# Autodesk Inventor assembly: Assembly-PCB alone
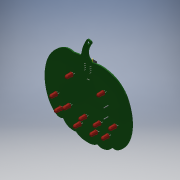
[picture p0: Inventor's stored thumbnail of the model, 180x180]
Saved by Autodesk Inventor 2018 (Build 220112000, 112)
## iProperties
Created: 2019-08-14
Part Number: Assembly-PCB alone
Document SubType Name: Assembly
Designer: Jamal Bouajjaj
Author: Jamal Bouajjaj
## iProperties of the stored document C_1206_3216Metric.iam
Created: 2019-10-04
Part Number: C_1206_3216Metric
Document SubType Name: Assembly
Designer: Electro707
Author: Electro707
## iProperties of the stored document SOLID.ipt
Created: 2019-10-04
Part Number: SOLID
Material: Generic
Document SubType Name: Modeling
Designer: Electro707
Density: 1 g/cm^3
Appearance: Default
Mass: 0.155302 g
Surface Area: 1.85065 cm^2
Volume: 0.155302 cm^3
Author: Electro707
## iProperties of the stored document BC2AAPC.iam
Created: 2019-10-04
Part Number: BC2AAPC
Document SubType Name: Assembly
Designer: Electro707
Author: Electro707
## iProperties of the stored document SOLID_2.ipt
Created: 2019-08-14
Part Number: SOLID_2
Material: Generic
Document SubType Name: Modeling
Designer: Jamal Bouajjaj
Density: 1 g/cm^3
Appearance: Default
Author: Jamal Bouajjaj
## iProperties of the stored document COMPOUND.ipt
Created: 2019-08-14
Part Number: COMPOUND
Material: Generic
Document SubType Name: Modeling
Designer: Jamal Bouajjaj
Density: 1 g/cm^3
Appearance: Default
Mass: 6.62606 g
Surface Area: 82.2116 cm^2
Volume: 6.62606 cm^3
Author: Jamal Bouajjaj
## iProperties of the stored document DIP-8_W7.62mm_Socket.iam
Created: 2019-08-14
Part Number: DIP-8_W7.62mm_Socket
Document SubType Name: Assembly
Designer: Jamal Bouajjaj
Author: Jamal Bouajjaj
## iProperties of the stored document SOLID_4.ipt
Created: 2019-08-14
Part Number: SOLID_4
Material: Generic
Document SubType Name: Modeling
Designer: Jamal Bouajjaj
Density: 1 g/cm^3
Appearance: Default
Mass: 0.075906 g
Surface Area: 1.25578 cm^2
Volume: 0.075906 cm^3
Author: Jamal Bouajjaj
## iProperties of the stored document SOLID_1.ipt
Created: 2019-08-14
Part Number: SOLID_1
Material: Generic
Document SubType Name: Modeling
Designer: Jamal Bouajjaj
Density: 1 g/cm^3
Appearance: Default
Author: Jamal Bouajjaj
## iProperties of the stored document DIP-8_W7.62mm.ipt
Company: FreeCAD
Created: 2017-03-07
Part Number: DIP-8_W7.62mm
Material: Generic
Description: model of DIP-8_W7.62mm
Document SubType Name: Modeling
Designer: Jamal Bouajjaj
Density: 1 g/cm^3
Appearance: Default
Mass: 0.184953 g
Surface Area: 2.97438 cm^2
Volume: 0.184953 cm^3
Sending System: kicad StepUp
Preprocessor: OCC
Title: DIP-8_W7.62mm.step
Author: kicad StepUp
## iProperties of the stored document SOLID_3.ipt
Created: 2019-08-14
Part Number: SOLID_3
Material: Generic
Document SubType Name: Modeling
Designer: Jamal Bouajjaj
Density: 1 g/cm^3
Appearance: Default
Mass: 0.20853 g
Surface Area: 4.37731 cm^2
Volume: 0.20853 cm^3
Author: Jamal Bouajjaj
## iProperties of the stored document PCB.iam
Created: 2019-10-04
Part Number: PCB
Description: KiCad electronic assembly
Document SubType Name: Assembly
Designer: Jamal Bouajjaj
Authority: Unknown
Company: A Company
Sending System: KiCad to STEP converter
Preprocessor: Open CASCADE STEP processor 6.9
Title: PCB.step
Author: An Author
## iProperties of the stored document R_1206_3216Metric.iam
Created: 2019-10-04
Part Number: R_1206_3216Metric
Document SubType Name: Assembly
Designer: Electro707
Author: Electro707
## iProperties of the stored document LED_D5.0mm.iam
Created: 2019-08-14
Part Number: LED_D5.0mm
Document SubType Name: Assembly
Designer: Jamal Bouajjaj
Author: Jamal Bouajjaj
## iProperties of the stored document TO-92_Inline.iam
Created: 2019-08-14
Part Number: TO-92_Inline
Document SubType Name: Assembly
Designer: Jamal Bouajjaj
Author: Jamal Bouajjaj
## iProperties of the stored document SOLID.ipt
Created: 2019-08-14
Part Number: SOLID
Material: Generic
Document SubType Name: Modeling
Designer: Jamal Bouajjaj
Density: 1 g/cm^3
Appearance: Default
Mass: 26.4084 g
Surface Area: 63.4129 cm^2
Volume: 26.4084 cm^3
Author: Jamal Bouajjaj
## Documents named in this file (20)
- **F:\Projects\UNH MakerSpace Kits\2019 - Halloween Event\Pumpkin\CAD-Inventor\Assembly-PCB alone.iam*LocalDocs*x243frfqbXew4u5clEhr01v13Hg*C_1206_3216Metric.iam
- **F:\Projects\UNH MakerSpace Kits\2019 - Halloween Event\Pumpkin\CAD-Inventor\Assembly-PCB alone.iam*LocalDocs*x1f3lsd2jFi21uesi0kw0jh2rMe*SOLID_2.ipt
- **F:\Projects\UNH MakerSpace Kits\2019 - Halloween Event\Pumpkin\CAD-Inventor\Assembly-PCB alone.iam*LocalDocs*x1ec2ztmoQijye4cbB0i4yov20a*SOLID.ipt
- **F:\Projects\UNH MakerSpace Kits\2019 - Halloween Event\Pumpkin\CAD-Inventor\Assembly-PCB alone.iam*LocalDocs*x03bjobyn0mvieqsn2uqwp0qkBf*BC2AAPC.iam
- **F:\Projects\UNH MakerSpace Kits\2019 - Halloween Event\Pumpkin\CAD-Inventor\Assembly-PCB alone.iam*LocalDocs*xTt1mklpdFqcruwk1B0ipitz2Qg*SOLID.ipt
- **F:\Projects\UNH MakerSpace Kits\2019 - Halloween Event\Pumpkin\CAD-Inventor\Assembly-PCB alone.iam*LocalDocs*xDucnimnbZ01bu3c2Gjb2coayUe*COMPOUND.ipt
- **F:\Projects\UNH MakerSpace Kits\2019 - Halloween Event\Pumpkin\CAD-Inventor\Assembly-PCB alone.iam*LocalDocs*xCuikmipqCcyeupooIhsm4atdUf*DIP-8_W7.62mm_Socket.iam
- **F:\Projects\UNH MakerSpace Kits\2019 - Halloween Event\Pumpkin\CAD-Inventor\Assembly-PCB alone.iam*LocalDocs*xE2pj1mn2Zvl3e4ctZa5bhgbzDh*SOLID_3.ipt
- **F:\Projects\UNH MakerSpace Kits\2019 - Halloween Event\Pumpkin\CAD-Inventor\Assembly-PCB alone.iam*LocalDocs*x35zwt44lF0yxuggtVufi3u0dRa*SOLID_4.ipt
- **F:\Projects\UNH MakerSpace Kits\2019 - Halloween Event\Pumpkin\CAD-Inventor\Assembly-PCB alone.iam*LocalDocs*xDmljyzhoUynuuwsrSorgzsefKc*SOLID_1.ipt
- **F:\Projects\UNH MakerSpace Kits\Haloween Board\2019\Pumpkin\CAD-Inventor\Assembly-PCB alone.iam*LocalDocs*xEdgsc3xdSn5neyc1Sb4f4rfzGg*DIP-8_W7.62mm.ipt
- **F:\Projects\UNH MakerSpace Kits\2019 - Halloween Event\Pumpkin\CAD-Inventor\Assembly-PCB alone.iam*LocalDocs*xKyv5v5xuIighelwx2z4bvtwzWf*PCB.iam
- **F:\Projects\UNH MakerSpace Kits\2019 - Halloween Event\Pumpkin\CAD-Inventor\Assembly-PCB alone.iam*LocalDocs*xLhgqzz5aUebjenwlV2x53kwiSd*TO-92_Inline.iam
- **F:\Projects\UNH MakerSpace Kits\2019 - Halloween Event\Pumpkin\CAD-Inventor\Assembly-PCB alone.iam*LocalDocs*xOxry2gm2K0mxejkvPmf12vio0d*LED_D5.0mm.iam
- **F:\Projects\UNH MakerSpace Kits\2019 - Halloween Event\Pumpkin\CAD-Inventor\Assembly-PCB alone.iam*LocalDocs*xFgilip1wCi2zuw4bKtyo4l5p4g*R_1206_3216Metric.iam
- F:\Projects\UNH MakerSpace Kits\2019 - Halloween Event\Pumpkin\GitHub Folder\CAD-Inventor\Assembly-PCB alone.iam
- **F:\Projects\UNH MakerSpace Kits\2019 - Halloween Event\Pumpkin\GitHub Folder\CAD-Inventor\Assembly-PCB alone.iam*LocalDocs*xKyv5v5xuIighelwx2z4bvtwzWf*PCB.iam
- **F:\Projects\UNH MakerSpace Kits\2019 - Halloween Event\Pumpkin\GitHub Folder\CAD-Inventor\Assembly-PCB alone.iam*LocalDocs*xEdgsc3xdSn5neyc1Sb4f4rfzGg*DIP-8_W7.62mm.ipt
- F:\Projects\UNH MakerSpace Kits\2019 - Halloween Event\Pumpkin\GitHub Folder\CAD-Inventor\DIP-8_W7.62mm.step
- F:\Projects\UNH MakerSpace Kits\2019 - Halloween Event\Pumpkin\GitHub Folder\CAD-Inventor\PCB.step
## Components (2 placed, 2 different names)
1. PCB:1 [sub-assembly] — Mate:1, Mate:14, Mate:15
2. DIP-8_W7.62mm:1 — Mate:1, Mate:2, Mate:3, Mate:4, Mate:5, Mate:6, Mate:7, Mate:8, Mate:9
## Relationships (15: Mate 15)
- Mate:1: PCB:1 ↔ DIP-8_W7.62mm:1
- Mate:2: DIP-8_W7.62mm:1
- Mate:3: DIP-8_W7.62mm:1
- Mate:4: DIP-8_W7.62mm:1
- Mate:5: DIP-8_W7.62mm:1
- Mate:6: DIP-8_W7.62mm:1
- Mate:7: DIP-8_W7.62mm:1
- Mate:8: DIP-8_W7.62mm:1
- Mate:9: DIP-8_W7.62mm:1
- Mate:10
- Mate:11
- Mate:12
- Mate:13
- Mate:14: PCB:1
- Mate:15: PCB:1
